# Autodesk Inventor assembly: eventide
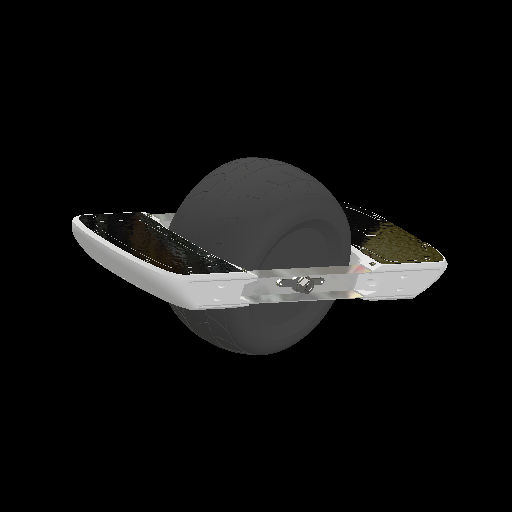
[picture p0: Inventor's stored thumbnail of the model, 512x512]
Saved by Autodesk Inventor 2025 (Build 290162000, 162)
## iProperties
Created: 2024-04-30
Part Number: eventide
Document SubType Name: Assembly
Designer: markm
Author: markm
## Documents named in this file (7)
- C:\Users\mark\OneDrive\Inventor\eventide\eventide.iam
- C:\Users\mark\OneDrive\Inventor\eventide\profile.ipt
- C:\Users\mark\OneDrive\Inventor\eventide\front\front.iam
- C:\Users\mark\OneDrive\Inventor\eventide\wheel\wheel.iam
- C:\Users\mark\OneDrive\Inventor\eventide\back\back.iam
- C:\Users\mark\OneDrive\Inventor\eventide\nut.ipt
- C:\Users\mark\OneDrive\Inventor\eventide\panel.ipt
## Components (9 placed, 6 different names)
1. profile:1 — Mate:1, Flush:1, Mate:2, Mate:4, Mate:7, Mate:8, Mate:9, Mate:15, Mate:19, Mate:22, Flush:10, Mate:29, Mate:30
2. profile:2 — Mate:1, Flush:1, Mate:4, Mate:26, Flush:13
3. front:1 [sub-assembly] — Mate:7, Flush:3, Mate:15, Mate:19, Mate:29
4. wheel:1 [sub-assembly] — Mate:3, Flush:2, Mate:20, Mate:23, Mate:24, Flush:11, Mate:25, Mate:27
5. back:1 [sub-assembly] — Mate:8, Mate:9, Mate:30
6. panel:1 — Mate:22, Mate:23, Mate:24, Flush:10
7. panel:2 — Mate:26, Mate:27, Flush:13, Mate:28
8. nut:1 — Mate:20, Flush:11
9. nut:2 — Mate:25, Mate:28
## Relationships (25: Mate 19, Flush 6)
- Mate:1: profile:1 ↔ profile:2
- Flush:1: profile:1 ↔ profile:2
- Mate:2: profile:1
- Mate:3: wheel:1
- Mate:4 (170 mm): profile:1 ↔ profile:2
- Flush:2: wheel:1
- Mate:7: profile:1 ↔ front:1
- Flush:3: front:1
- Mate:8: profile:1 ↔ back:1
- Mate:9: profile:1 ↔ back:1
- Mate:15: profile:1 ↔ front:1
- Mate:19: profile:1 ↔ front:1
- Mate:20: wheel:1 ↔ nut:1
- Mate:22: profile:1 ↔ panel:1
- Mate:23: wheel:1 ↔ panel:1
- Mate:24: wheel:1 ↔ panel:1
- Flush:10: profile:1 ↔ panel:1
- Flush:11: wheel:1 ↔ nut:1
- Mate:25: wheel:1 ↔ nut:2
- Mate:26: profile:2 ↔ panel:2
- Mate:27: wheel:1 ↔ panel:2
- Flush:13: profile:2 ↔ panel:2
- Mate:28: panel:2 ↔ nut:2
- Mate:29: profile:1 ↔ front:1
- Mate:30: profile:1 ↔ back:1
